# Autodesk Inventor assembly: ProtectionCatapult
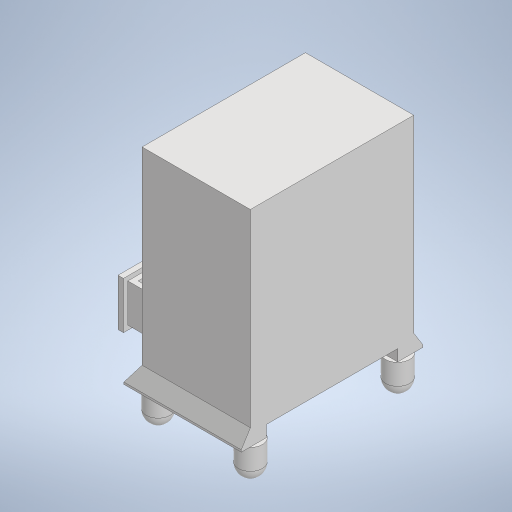
[picture p0: Inventor's stored thumbnail of the model, 512x512]
Saved by Autodesk Inventor 2024 (Build 280153000, 153)
## iProperties
Created: 2025-02-23
Part Number: ProtectionCatapult
Document SubType Name: Assembly
Designer: sergi
Author: sergi
## Documents named in this file (4)
- C:\Users\sergi\OneDrive\Escritorio\Projects\16. Protection catapult\Inventor\ProtectionCatapult.iam
- C:\Users\sergi\OneDrive\Escritorio\Projects\16. Protection catapult\Inventor\Cajon.ipt
- C:\Users\sergi\OneDrive\Escritorio\Projects\16. Protection catapult\Inventor\Comoda.ipt
- C:\Users\sergi\OneDrive\Escritorio\NEMA17_Mirror.A.0.ipt
## Components (6 placed, 3 different names)
1. Cajon:1 — Coincidencia:1, Coincidencia:2
2. Comoda:1 — Coincidencia:1, Coincidencia:2, Coincidencia:3, Coincidencia:4, Coincidencia:5, Coincidencia:6, Coincidencia:7, Coincidencia:8, Coincidencia:9, Coincidencia:10, Coincidencia:11, Coincidencia:12, Nivelación:1, Nivelación:2
3. Cajon:2 — Coincidencia:3, Coincidencia:4, Coincidencia:5
4. Cajon:3 — Coincidencia:6, Coincidencia:7, Coincidencia:8
5. NEMA17_Mirror.A.0:1 — Coincidencia:9, Coincidencia:10, Nivelación:2
6. NEMA17_Mirror.A.0:2 — Coincidencia:11, Coincidencia:12, Nivelación:1
## Relationships (14: Mate 12, Flush 2)
- Coincidencia:1 [Mate]: Cajon:1 ↔ Comoda:1
- Coincidencia:2 [Mate] (2.5 mm): Cajon:1 ↔ Comoda:1
- Coincidencia:3 [Mate]: Comoda:1 ↔ Cajon:2
- Coincidencia:4 [Mate] (2.5 mm): Comoda:1 ↔ Cajon:2
- Coincidencia:5 [Mate]: Comoda:1 ↔ Cajon:2
- Coincidencia:6 [Mate]: Comoda:1 ↔ Cajon:3
- Coincidencia:7 [Mate]: Comoda:1 ↔ Cajon:3
- Coincidencia:8 [Mate] (2.5 mm): Comoda:1 ↔ Cajon:3
- Coincidencia:9 [Mate]: Comoda:1 ↔ NEMA17_Mirror.A.0:1
- Coincidencia:10 [Mate]: Comoda:1 ↔ NEMA17_Mirror.A.0:1
- Coincidencia:11 [Mate]: Comoda:1 ↔ NEMA17_Mirror.A.0:2
- Coincidencia:12 [Mate]: Comoda:1 ↔ NEMA17_Mirror.A.0:2
- Nivelación:1 [Flush]: Comoda:1 ↔ NEMA17_Mirror.A.0:2
- Nivelación:2 [Flush]: Comoda:1 ↔ NEMA17_Mirror.A.0:1
